# Autodesk Inventor assembly: m0.5z80
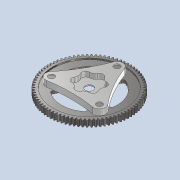
[picture p0: Inventor's stored thumbnail of the model, 180x180]
Saved by Autodesk Inventor 2020.4 (Build 244396000, 396)
## iProperties
Created: 2021-04-23
Part Number: m0.5z80
Document SubType Name: Assembly
Designer: happy
Author: happy
## Documents named in this file (4)
- C:\Users\happy\OneDrive\ドキュメント\賢一ファイル\SRDC\試作10-2\アームギア\m0.5z80.iam
- C:\Users\happy\OneDrive\ドキュメント\賢一ファイル\SRDC\試作10-2\ギア\歯車m0.5,z80.ipt
- C:\Users\happy\OneDrive\ドキュメント\賢一ファイル\SRDC\試作10-2\アームギア\m0.5z80接続部品.ipt
- C:\Users\happy\OneDrive\ドキュメント\賢一ファイル\SRDC\試作10-2\ねじ\M3L4　超極低頭.ipt
## Components (5 placed, 3 different names)
1. 歯車m0.5,z80:1 — 挿入:1, 挿入:2, 挿入:3, 挿入:4, 挿入:5
2. m0.5z80接続部品:1 — 挿入:1, 挿入:2
3. M3L4　超極低頭:1 — 挿入:3
4. M3L4　超極低頭:2 — 挿入:4
5. M3L4　超極低頭:3 — 挿入:5
## Relationships (5: Insert 5)
- 挿入:1 [Insert]: 歯車m0.5,z80:1 ↔ m0.5z80接続部品:1
- 挿入:2 [Insert]: 歯車m0.5,z80:1 ↔ m0.5z80接続部品:1
- 挿入:3 [Insert]: 歯車m0.5,z80:1 ↔ M3L4　超極低頭:1
- 挿入:4 [Insert]: 歯車m0.5,z80:1 ↔ M3L4　超極低頭:2
- 挿入:5 [Insert]: 歯車m0.5,z80:1 ↔ M3L4　超極低頭:3
